# Autodesk Inventor assembly: ASY PNS-0210 frame right floor
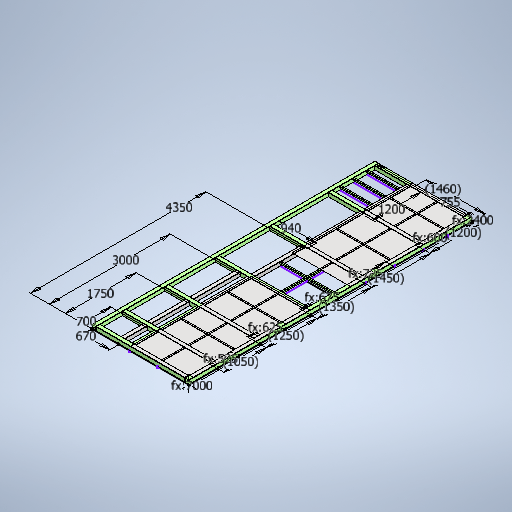
[picture p0: Inventor's stored thumbnail of the model, 512x512]
Saved by Autodesk Inventor 2025 (Build 290162010, 162A)
## iProperties
Created: 2025-03-15
Part Number: ASY PNS-0210 frame right floor
Document SubType Name: Assembly
Designer: admin
Mass: 658050 g
Surface Area: 604170 cm^2
Volume: 83312 cm^3
Density: 7.89861 g/cm^3
_SolveAssemblyDoc: Frame Generator Solve Assembly
_Version: 25.0.0
Author: admin
## Documents named in this file (4)
- C:\Users\admin\YandexDisk-badmisterfox\home pc\Inventor\PNS-Panaevsk\ASY PNS-0210 frame right floor.iam
- C:\Users\admin\YandexDisk-badmisterfox\home pc\Inventor\PNS-Panaevsk\PNS-0210 frame right floor Sketch.ipt
- C:\Users\admin\YandexDisk-badmisterfox\home pc\Inventor\PNS-Panaevsk\ASY PNS-0210 frame right floor\Frame\Frame 1742033625963.iam
- C:\Users\admin\YandexDisk-badmisterfox\home pc\Inventor\PNS-Panaevsk\PNS-0111 floor sheet 2.ipt
## Components (4 placed, 3 different names)
1. PNS-0210 frame right floor Sketch:1
2. PNS-0111 floor sheet 2:2 — Rigid:1
3. Frame 1742033625963:1 [sub-assembly] — Rigid:1, Rigid:2
4. PNS-0111 floor sheet 2:3 — Rigid:2
## Relationships (2: WeldJoint 2)
- Rigid:1 [WeldJoint] (-116 mm): PNS-0111 floor sheet 2:2 ↔ Frame 1742033625963:1
- Rigid:2 [WeldJoint] (116 mm): Frame 1742033625963:1 ↔ PNS-0111 floor sheet 2:3
